# Autodesk Inventor assembly: MPU
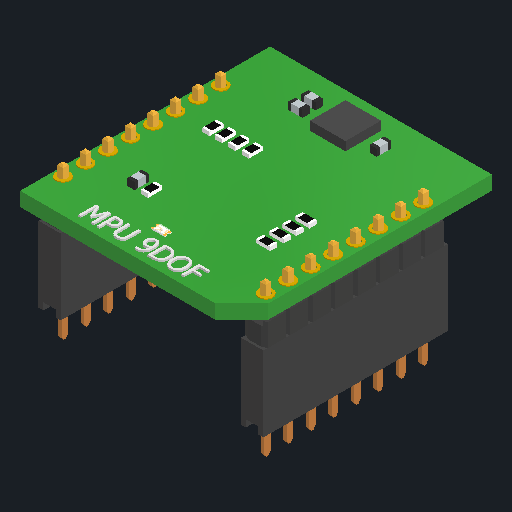
[picture p0: Inventor's stored thumbnail of the model, 512x512]
Saved by Autodesk Inventor 2022 (Build 260153000, 153)
## iProperties
Created: 2022-03-19
Part Number: MPU
Document SubType Name: Assembly
Designer: dvorakj
Author: dvorakj
## Documents named in this file (7)
- C:\Users\dvorakj\Documents\Inventor\Bakalarka\Clicks\MPU\MPU.iam
- C:\Users\dvorakj\Documents\Inventor\Bakalarka\Clicks\MPU\GPS_PCB.ipt
- C:\Users\dvorakj\Documents\Inventor\Bakalarka\Clicks\MPU\LED\STP_WL-SMCW_150060xx75020 (rev1).iam
- C:\Users\dvorakj\Documents\Inventor\Bakalarka\Clicks\MPU\MPU_chip.ipt
- C:\Users\dvorakj\Documents\Inventor\Bakalarka\Clicks\Pin Header\61300811121 (rev1).iam
- C:\Users\dvorakj\Documents\Inventor\Bakalarka\Common\RES\Resistor_0603.iam
- C:\Users\dvorakj\Documents\Inventor\Bakalarka\Common\CAP\Download_STP_8850122060xx (rev1).iam
## Components (18 placed, 6 different names)
1. GPS_PCB:1 — Mate:1, Flush:1, Mate:2, Mate:3, Mate:4, Mate:5, Mate:6
2. STP_WL-SMCW_150060xx75020 (rev1):1 [sub-assembly] — Mate:1
3. MPU_chip:1 — Flush:1
4. 61300811121 (rev1):1 [sub-assembly] — Mate:2, Mate:4
5. 61300811121 (rev1):2 [sub-assembly] — Mate:3, Mate:5
6. Resistor_0603:1 [sub-assembly] — Flush:4, Flush:17
7. Resistor_0603:2 [sub-assembly] — Flush:5, Flush:17, Flush:18
8. Resistor_0603:3 [sub-assembly] — Flush:6, Flush:18, Flush:19
9. Resistor_0603:4 [sub-assembly] — Flush:7, Flush:8, Flush:9, Flush:19
10. Resistor_0603:5 [sub-assembly] — Flush:9, Flush:10, Flush:15, Flush:16
11. Resistor_0603:6 [sub-assembly] — Flush:10, Flush:11, Flush:14, Flush:15
12. Resistor_0603:7 [sub-assembly] — Flush:11, Flush:13, Flush:14
13. Resistor_0603:8 [sub-assembly] — Flush:8, Flush:16
14. Resistor_0603:9 [sub-assembly] — Flush:12, Flush:13, Mate:6, Flush:20
15. Download_STP_8850122060xx (rev1):1 [sub-assembly] — Flush:2, Flush:3, Flush:21
16. Download_STP_8850122060xx (rev1):2 [sub-assembly] — Flush:2, Flush:4, Flush:5, Flush:6, Flush:7, Flush:21
17. Download_STP_8850122060xx (rev1):3 [sub-assembly] — Flush:3, Flush:20
18. Download_STP_8850122060xx (rev1):4 [sub-assembly] — Flush:12
## Relationships (27: Flush 21, Mate 6)
- Mate:1: GPS_PCB:1 ↔ STP_WL-SMCW_150060xx75020 (rev1):1
- Flush:1: GPS_PCB:1 ↔ MPU_chip:1
- Mate:2: GPS_PCB:1 ↔ 61300811121 (rev1):1
- Mate:3: GPS_PCB:1 ↔ 61300811121 (rev1):2
- Mate:4: GPS_PCB:1 ↔ 61300811121 (rev1):1
- Mate:5: GPS_PCB:1 ↔ 61300811121 (rev1):2
- Flush:2: Download_STP_8850122060xx (rev1):1 ↔ Download_STP_8850122060xx (rev1):2
- Flush:3: Download_STP_8850122060xx (rev1):1 ↔ Download_STP_8850122060xx (rev1):3
- Flush:4: Resistor_0603:1 ↔ Download_STP_8850122060xx (rev1):2
- Flush:5: Resistor_0603:2 ↔ Download_STP_8850122060xx (rev1):2
- Flush:6: Resistor_0603:3 ↔ Download_STP_8850122060xx (rev1):2
- Flush:7: Resistor_0603:4 ↔ Download_STP_8850122060xx (rev1):2
- Flush:8: Resistor_0603:4 ↔ Resistor_0603:8
- Flush:9: Resistor_0603:4 ↔ Resistor_0603:5
- Flush:10: Resistor_0603:5 ↔ Resistor_0603:6
- Flush:11: Resistor_0603:6 ↔ Resistor_0603:7
- Flush:12: Resistor_0603:9 ↔ Download_STP_8850122060xx (rev1):4
- Flush:13: Resistor_0603:7 ↔ Resistor_0603:9
- Mate:6: GPS_PCB:1 ↔ Resistor_0603:9
- Flush:14: Resistor_0603:6 ↔ Resistor_0603:7
- Flush:15: Resistor_0603:5 ↔ Resistor_0603:6
- Flush:16: Resistor_0603:5 ↔ Resistor_0603:8
- Flush:17: Resistor_0603:1 ↔ Resistor_0603:2
- Flush:18: Resistor_0603:2 ↔ Resistor_0603:3
- Flush:19: Resistor_0603:3 ↔ Resistor_0603:4
- Flush:20: Resistor_0603:9 ↔ Download_STP_8850122060xx (rev1):3
- Flush:21: Download_STP_8850122060xx (rev1):1 ↔ Download_STP_8850122060xx (rev1):2
